# Autodesk Inventor assembly: RobotFrame
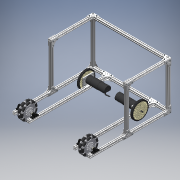
[picture p0: Inventor's stored thumbnail of the model, 180x180]
Saved by Autodesk Inventor 2017.3 (Build 213256000, 256)
## iProperties
Created: 2018-01-04
Part Number: RobotFrame
Document SubType Name: Assembly
Designer: pranav
Author: pranav
## iProperties of the stored document REV-41-1432.ipt
Created: 2017-04-10
Part Number: REV-41-1432
Material: Generic
Document SubType Name: Modeling
Designer: pranav
Density: 1 g/cm^3
Appearance: Default
Sending System: Autodesk Translation Framework v5.2.0.2920
Preprocessor: ST-DEVELOPER v16.5
Title: E:/Dropbox/REV Robotics/STEP Files/REV-41-1432.step
## iProperties of the stored document REV-41-1301.ipt
Created: 2016-09-02
Part Number: REV-41-1301
Material: Generic
Description: STEP AP203
Document SubType Name: Modeling
Designer: pranav
Density: 1 g/cm^3
Appearance: Default
Sending System: SolidWorks 2015
Preprocessor: SwSTEP 2.0
Title: REV-41-1301.STEP
Revision Number: ANY
## iProperties of the stored document REV-41-1347.ipt
Created: 2016-09-04
Part Number: REV-41-1347
Material: Generic
Description: STEP AP203
Document SubType Name: Modeling
Designer: pranav
Density: 1 g/cm^3
Appearance: Default
Sending System: SolidWorks 2015
Preprocessor: SwSTEP 2.0
Title: REV-41-1347_Default.step
Revision Number: ANY
## iProperties of the stored document REV-41-1431.ipt
Created: 2017-04-10
Part Number: REV-41-1431
Material: Generic
Document SubType Name: Modeling
Designer: pranav
Density: 1 g/cm^3
Appearance: Default
Sending System: Autodesk Translation Framework v5.2.0.2920
Preprocessor: ST-DEVELOPER v16.5
Title: E:/Dropbox/REV Robotics/STEP Files/REV-41-1431.step
## Documents named in this file (16)
- **C:\Users\pranav\Documents\Inventor\REV-Robot-CAD\RobotFrame.iam*LocalDocs*x4xurmugoHsr3ubcqL1pqt4jsKh*REV-41-1432.ipt
- **C:\Users\pranav\Documents\Inventor\REV-Robot-CAD\RobotFrame.iam*LocalDocs*x3mmmsddaKdzrefwn3gzdw4fjCd*REV-41-1301.ipt
- **C:\Users\pranav\Documents\Inventor\REV-Robot-CAD\RobotFrame.iam*LocalDocs*xEx30atbkKgg2emcoTihhwmmkQg*REV-41-1347.ipt
- **C:\Users\pranav\Documents\Inventor\REV-Robot-CAD\RobotFrame.iam*LocalDocs*xFl3mf32hAd4qexc0Tvxp5ln1Fc*REV-41-1431.ipt
- C:\Users\pranav\Documents\Inventor\REV-Robot-CAD\RobotFrame.iam
- C:\Users\pranav\Documents\Inventor\REV-Robot-CAD\3D-Metal-Corner.iam
- C:\Users\pranav\Documents\Inventor\REV-Robot-CAD\T-Metal-Brace.iam
- C:\Users\pranav\Documents\Inventor\REV-Robot-CAD\90-Degree-Metal-Brace.iam
- C:\Users\pranav\Documents\Inventor\REV-Robot-CAD\HD-Motor-Mount.iam
- C:\Users\pranav\Documents\Inventor\REV-Robot-CAD\REV-41-1354.ipt
- C:\Users\pranav\Documents\Inventor\REV-Robot-CAD\Bearing-Pillow-Block-Short-Through-Bore.iam
- C:\Users\pranav\Documents\Inventor\REV-Robot-CAD\Double-Stack-Omni-Wheels.iam
- C:\Users\pranav\Documents\Inventor\REV-Robot-CAD\REV Robotics\REV Robotics CAD\REV-41-1432.step
- C:\Users\pranav\Documents\Inventor\REV-Robot-CAD\REV Robotics\REV Robotics CAD\REV-41-1431.step
- C:\Users\pranav\Documents\Inventor\REV-Robot-CAD\REV Robotics\REV Robotics CAD\REV-41-1301.STEP
- C:\Users\pranav\Documents\Inventor\REV-Robot-CAD\REV Robotics\REV Robotics CAD\REV-41-1347.step
## Components (36 placed, 11 different names)
1. REV-41-1432:1 — Mate:1, Flush:1, Flush:2, Mate:2, Flush:3, Flush:4, Mate:14, Mate:15, Mate:17, Mate:18, Mate:26, Flush:27, Mate:28, Flush:28, Mate:30, Flush:29, Flush:31
2. REV-41-1432:2 — Mate:2, Flush:3, Flush:4, Mate:19, Flush:26, Mate:27, Mate:44, Mate:46, Flush:43
3. REV-41-1432:4 — Mate:6, Flush:11, Flush:12, Mate:7, Flush:13, Flush:14, Mate:11, Mate:20, Mate:22
4. REV-41-1432:5 — Mate:1, Flush:1, Flush:2, Mate:16, Flush:24, Mate:29, Mate:39, Mate:40, Mate:60, Flush:38
5. REV-41-1431:1 — Mate:7, Flush:13, Flush:14, Mate:10, Flush:20, Mate:12, Mate:13
6. REV-41-1431:2 — Mate:6, Flush:11, Flush:12, Mate:21, Mate:23, Flush:21, Flush:22, Mate:49, Flush:37
7. 3D-Metal-Corner:1 [sub-assembly] — Mate:17, Mate:18, Mate:19, Mate:47, Mate:48
8. 3D-Metal-Corner:2 [sub-assembly] — Mate:14, Mate:15, Mate:16, Mate:41, Mate:42
9. 3D-Metal-Corner:3 [sub-assembly] — Mate:11, Mate:12, Mate:13
10. 3D-Metal-Corner:4 [sub-assembly] — Mate:20, Mate:21, Mate:22
11. T-Metal-Brace:1 [sub-assembly] — Flush:24, Mate:43, Flush:35
12. T-Metal-Brace:2 [sub-assembly] — Flush:26, Mate:45, Flush:36
13. 90-Degree-Metal-Brace:1 [sub-assembly] — Mate:10, Flush:20
14. 90-Degree-Metal-Brace:2 [sub-assembly] — Mate:23, Flush:21, Flush:22
15. REV-41-1432:11 — Mate:28, Flush:28, Mate:29, Flush:30, Mate:32, Flush:33, Flush:41
16. REV-41-1432:12 — Mate:26, Mate:27, Flush:27, Mate:31, Flush:32, Mate:34, Flush:34, Flush:42
17. T-Metal-Brace:3 [sub-assembly] — Mate:30, Flush:29, Flush:30, Mate:33
18. T-Metal-Brace:4 [sub-assembly] — Mate:31, Flush:31, Flush:32, Mate:35
19. HD-Motor-Mount:1 [sub-assembly] — Mate:32, Flush:33, Mate:33, Mate:52, Mate:53
20. HD-Motor-Mount:2 [sub-assembly] — Mate:34, Flush:34, Mate:35, Mate:50, Mate:51
21. REV-41-1301:1 — Mate:52, Mate:53, Mate:58, Mate:59
22. REV-41-1301:2 — Mate:50, Mate:51, Mate:56, Mate:57
23. REV-41-1431:3 — Mate:39, Mate:43, Flush:35, Mate:49, Flush:37
24. REV-41-1431:4 — Mate:40, Mate:41, Mate:42
25. REV-41-1431:5 — Mate:44, Mate:45, Flush:36
26. REV-41-1431:6 — Mate:46, Mate:47, Mate:48
27. REV-41-1354:1 — Mate:56, Mate:57
28. REV-41-1354:2 — Mate:58, Mate:59
29. Bearing-Pillow-Block-Short-Through-Bore:1 [sub-assembly] — Mate:60, Flush:38, Mate:61, Flush:44
30. Bearing-Pillow-Block-Short-Through-Bore:4 [sub-assembly] — Flush:41, Mate:64
31. Bearing-Pillow-Block-Short-Through-Bore:5 [sub-assembly] — Flush:42
32. Bearing-Pillow-Block-Short-Through-Bore:6 [sub-assembly] — Flush:43, Flush:45, Mate:62, Mate:66
33. REV-41-1347:1 — Mate:61, Flush:44, Mate:63
34. REV-41-1347:2 — Flush:45, Mate:62, Mate:65
35. Double-Stack-Omni-Wheels:1 [sub-assembly] — Mate:65, Mate:66
36. Double-Stack-Omni-Wheels:2 [sub-assembly] — Mate:63, Mate:64
## Relationships (84: Mate 54, Flush 30)
- Mate:1: REV-41-1432:1 ↔ REV-41-1432:5
- Flush:1: REV-41-1432:1 ↔ REV-41-1432:5
- Flush:2: REV-41-1432:1 ↔ REV-41-1432:5
- Mate:2: REV-41-1432:1 ↔ REV-41-1432:2
- Flush:3: REV-41-1432:1 ↔ REV-41-1432:2
- Flush:4: REV-41-1432:1 ↔ REV-41-1432:2
- Mate:6: REV-41-1432:4 ↔ REV-41-1431:2
- Flush:11: REV-41-1432:4 ↔ REV-41-1431:2
- Flush:12: REV-41-1432:4 ↔ REV-41-1431:2
- Mate:7: REV-41-1432:4 ↔ REV-41-1431:1
- Flush:13: REV-41-1432:4 ↔ REV-41-1431:1
- Flush:14: REV-41-1432:4 ↔ REV-41-1431:1
- Mate:10: REV-41-1431:1 ↔ 90-Degree-Metal-Brace:1
- Flush:20: REV-41-1431:1 ↔ 90-Degree-Metal-Brace:1
- Mate:11: REV-41-1432:4 ↔ 3D-Metal-Corner:3
- Mate:12: REV-41-1431:1 ↔ 3D-Metal-Corner:3
- Mate:13: REV-41-1431:1 ↔ 3D-Metal-Corner:3
- Mate:14: REV-41-1432:1 ↔ 3D-Metal-Corner:2
- Mate:15: REV-41-1432:1 ↔ 3D-Metal-Corner:2
- Mate:16: REV-41-1432:5 ↔ 3D-Metal-Corner:2
- Mate:17: REV-41-1432:1 ↔ 3D-Metal-Corner:1
- Mate:18: REV-41-1432:1 ↔ 3D-Metal-Corner:1
- Mate:19: REV-41-1432:2 ↔ 3D-Metal-Corner:1
- Mate:20: REV-41-1432:4 ↔ 3D-Metal-Corner:4
- Mate:21: REV-41-1431:2 ↔ 3D-Metal-Corner:4
- Mate:22: REV-41-1432:4 ↔ 3D-Metal-Corner:4
- Mate:23: REV-41-1431:2 ↔ 90-Degree-Metal-Brace:2
- Flush:21: REV-41-1431:2 ↔ 90-Degree-Metal-Brace:2
- Flush:22: REV-41-1431:2 ↔ 90-Degree-Metal-Brace:2
- Flush:24: REV-41-1432:5 ↔ T-Metal-Brace:1
- Flush:26: REV-41-1432:2 ↔ T-Metal-Brace:2
- Mate:26: REV-41-1432:1 ↔ REV-41-1432:12
- Mate:27 (63.5 mm): REV-41-1432:2 ↔ REV-41-1432:12
- Flush:27: REV-41-1432:1 ↔ REV-41-1432:12
- Mate:28: REV-41-1432:1 ↔ REV-41-1432:11
- Flush:28: REV-41-1432:1 ↔ REV-41-1432:11
- Mate:29 (63.5 mm): REV-41-1432:5 ↔ REV-41-1432:11
- Mate:30: REV-41-1432:1 ↔ T-Metal-Brace:3
- Flush:29: REV-41-1432:1 ↔ T-Metal-Brace:3
- Flush:30: REV-41-1432:11 ↔ T-Metal-Brace:3
- Mate:31: REV-41-1432:12 ↔ T-Metal-Brace:4
- Flush:31: REV-41-1432:1 ↔ T-Metal-Brace:4
- Flush:32: REV-41-1432:12 ↔ T-Metal-Brace:4
- Mate:32: REV-41-1432:11 ↔ HD-Motor-Mount:1
- Flush:33: REV-41-1432:11 ↔ HD-Motor-Mount:1
- Mate:33 (38.1 mm): T-Metal-Brace:3 ↔ HD-Motor-Mount:1
- Mate:34: REV-41-1432:12 ↔ HD-Motor-Mount:2
- Flush:34: REV-41-1432:12 ↔ HD-Motor-Mount:2
- Mate:35 (38.1 mm): T-Metal-Brace:4 ↔ HD-Motor-Mount:2
- Mate:39: REV-41-1432:5 ↔ REV-41-1431:3
- Mate:40: REV-41-1432:5 ↔ REV-41-1431:4
- Mate:41: 3D-Metal-Corner:2 ↔ REV-41-1431:4
- Mate:42: 3D-Metal-Corner:2 ↔ REV-41-1431:4
- Mate:43: T-Metal-Brace:1 ↔ REV-41-1431:3
- Flush:35: T-Metal-Brace:1 ↔ REV-41-1431:3
- Mate:44: REV-41-1432:2 ↔ REV-41-1431:5
- Mate:45: T-Metal-Brace:2 ↔ REV-41-1431:5
- Flush:36: T-Metal-Brace:2 ↔ REV-41-1431:5
- Mate:46: REV-41-1432:2 ↔ REV-41-1431:6
- Mate:47: 3D-Metal-Corner:1 ↔ REV-41-1431:6
- Mate:48: 3D-Metal-Corner:1 ↔ REV-41-1431:6
- Mate:49: REV-41-1431:2 ↔ REV-41-1431:3
- Flush:37: REV-41-1431:2 ↔ REV-41-1431:3
- Mate:50: HD-Motor-Mount:2 ↔ REV-41-1301:2
- Mate:51: HD-Motor-Mount:2 ↔ REV-41-1301:2
- Mate:52: HD-Motor-Mount:1 ↔ REV-41-1301:1
- Mate:53: HD-Motor-Mount:1 ↔ REV-41-1301:1
- Mate:56: REV-41-1301:2 ↔ REV-41-1354:1
- Mate:57: REV-41-1301:2 ↔ REV-41-1354:1
- Mate:58: REV-41-1301:1 ↔ REV-41-1354:2
- Mate:59: REV-41-1301:1 ↔ REV-41-1354:2
- Mate:60: REV-41-1432:5 ↔ Bearing-Pillow-Block-Short-Through-Bore:1
- Flush:38: REV-41-1432:5 ↔ Bearing-Pillow-Block-Short-Through-Bore:1
- Flush:41: REV-41-1432:11 ↔ Bearing-Pillow-Block-Short-Through-Bore:4
- Flush:42: REV-41-1432:12 ↔ Bearing-Pillow-Block-Short-Through-Bore:5
- Flush:43: REV-41-1432:2 ↔ Bearing-Pillow-Block-Short-Through-Bore:6
- Mate:61: Bearing-Pillow-Block-Short-Through-Bore:1 ↔ REV-41-1347:1
- Flush:44: Bearing-Pillow-Block-Short-Through-Bore:1 ↔ REV-41-1347:1
- Flush:45: Bearing-Pillow-Block-Short-Through-Bore:6 ↔ REV-41-1347:2
- Mate:62: Bearing-Pillow-Block-Short-Through-Bore:6 ↔ REV-41-1347:2
- Mate:63: REV-41-1347:1 ↔ Double-Stack-Omni-Wheels:2
- Mate:64 (6.6923 mm): Bearing-Pillow-Block-Short-Through-Bore:4 ↔ Double-Stack-Omni-Wheels:2
- Mate:65: REV-41-1347:2 ↔ Double-Stack-Omni-Wheels:1
- Mate:66 (6.6923 mm): Bearing-Pillow-Block-Short-Through-Bore:6 ↔ Double-Stack-Omni-Wheels:1
## Named parameters: WheelExtrusionOffset = 63.5 mm
